# Autodesk Inventor assembly: Assembly1
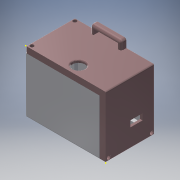
[picture p0: Inventor's stored thumbnail of the model, 180x180]
Saved by Autodesk Inventor 2019 (Build 230136000, 136)
## iProperties
Created: 2019-02-08
Part Number: Assembly1
Document SubType Name: Assembly
Designer: darky
Author: darky
## Documents named in this file (3)
- C:\Users\darky\Documents\Universidad\10 Redes Wireless y Moviles\Proyecto Final con ESP32\Assembly1.iam
- C:\Users\darky\Documents\Universidad\10 Redes Wireless y Moviles\Proyecto Final con ESP32\Part1.ipt
- C:\Users\darky\Documents\Universidad\10 Redes Wireless y Moviles\Proyecto Final con ESP32\Part3.ipt
## Components (2 placed, 2 different names)
1. Part1:1 — Rigid:1
2. Part3:1 — Rigid:1
## Relationships (1: WeldJoint 1)
- Rigid:1 [WeldJoint]: Part1:1 ↔ Part3:1
